# Autodesk Inventor assembly: ASY HPR 200  Frame
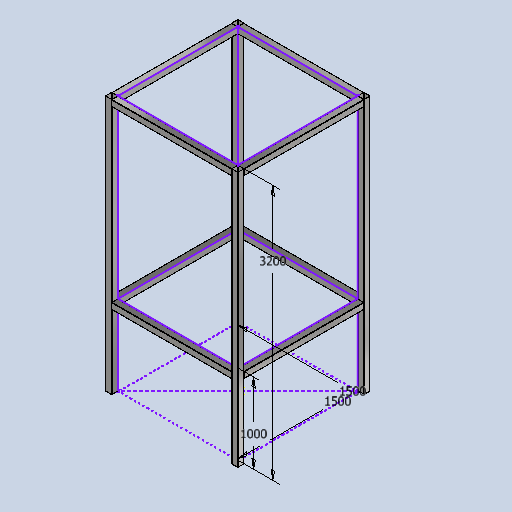
[picture p0: Inventor's stored thumbnail of the model, 512x512]
Saved by Autodesk Inventor 2025.1 (Build 291241020, 241B)
## iProperties
_SolveAssemblyDoc: Frame Generator Solve Assembly
_Version: 25.0.0
Created: 2024-11-03
Part Number: ASY HPR 200  Frame
Document SubType Name: Assembly
Designer: admin
Author: admin
## Documents named in this file (3)
- C:\Users\user\YandexDisk-badmisterfox\домашниий пк\Inventor\NDM-VOS_powder_hopper\ASY HPR 200  Frame.iam
- C:\Users\user\YandexDisk-badmisterfox\домашниий пк\Inventor\NDM-VOS_powder_hopper\NDM-VOS Рама Эскиз.ipt
- C:\Users\user\YandexDisk-badmisterfox\домашниий пк\Inventor\NDM-VOS_powder_hopper\ASY HPR 200  Frame\Frame\Frame 1730655523663.iam
## Components (2 placed, 2 different names)
1. NDM-VOS Рама Эскиз:1 — Mate:1, Flush:5, Flush:4
2. Frame 1730655523663:1 [sub-assembly]
## Relationships (3: Flush 2, Mate 1)
- Mate:1: NDM-VOS Рама Эскиз:1
- Flush:5: NDM-VOS Рама Эскиз:1
- Flush:4: NDM-VOS Рама Эскиз:1
